# Autodesk Inventor assembly: OBG-Elektronik
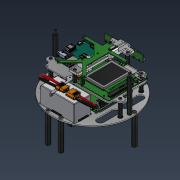
[picture p0: Inventor's stored thumbnail of the model, 180x180]
Saved by Autodesk Inventor 2022.1 (Build 261234020, 234B)
## iProperties
Part Number: OBG-Elektronik
Material: Generisch
Document SubType Name: Assembly
Designer: rYan
Mass: 726.974 g
Surface Area: 2264.16 cm^2
Volume: 285.444 cm^3
Density: 2.54682 g/cm^3
Author: rYan
## Documents named in this file (16)
- D:\TIGERsGIT\Hardware\mechanik\2020\Inventor\Robot\Electronics\OBG-Elektronik.iam
- D:\TIGERsGIT\Hardware\mechanik\2020\Inventor\Robot\Electronics\Mittelplatte.ipt
- D:\TIGERsGIT\Hardware\mechanik\2019\Inventor\Kaufteile\Abstandsbolzen Typ A.ipt
- D:\TIGERsGIT\Hardware\mechanik\2020\Inventor\Inhaltscenter\de-DE\DIN 7984\DIN 7984 - M4 x 6.ipt
- D:\TIGERsGIT\Hardware\mechanik\2020\Inventor\Purchased Parts\Abstandsbolzen Typ A M4 60mm SW8.ipt
- D:\TIGERsGIT\Hardware\mechanik\2020\Inventor\Robot\Electronics\MG-Powerboard.iam
- D:\TIGERsGIT\Hardware\mechanik\2019\Inventor\Kaufteile\Abstandsbolzen Typ B.ipt
- D:\TIGERsGIT\Hardware\mechanik\2020\Inventor\Robot\Electronics\UBG-Compute Layer.iam
- D:\TIGERsGIT\Hardware\mechanik\2020\Inventor\Purchased Parts\Abstandsbolzen Typ B M4 70mm.ipt
- D:\TIGERsGIT\Hardware\mechanik\2020\Inventor\Purchased Parts\MG-Akku 6S1P.iam
- D:\TIGERsGIT\Hardware\mechanik\2020\Inventor\Robot\Electronics\Akkuhalter.ipt
- D:\TIGERsGIT\Hardware\mechanik\2020\Inventor\Purchased Parts\Gummitülle 3mm.ipt
- D:\TIGERsGIT\Hardware\mechanik\2020\Inventor\Inhaltscenter\de-DE\ISO 4762(2)\ISO 4762 - M2 x 6ISO.ipt
- D:\TIGERsGIT\Hardware\mechanik\2020\Inventor\Robot\Electronics\UBG-Kamera mit Halter geneigt.iam
- D:\TIGERsGIT\Hardware\mechanik\2020\Inventor\Inhaltscenter\de-DE\DIN 7984\DIN 7984 - M3 x 5.ipt
- D:\TIGERsGIT\Hardware\mechanik\2020\Inventor\Inhaltscenter\de-DE\ISO 10642(1)\ISO 10642 - M3 x  8.ipt
## Components (32 placed, 13 different names)
1. Mittelplatte:1 — Einfügen:1, Einfügen:3, Einfügen:4, Einfügen:6, Einfügen:7, Einfügen:8, Fluchtend:1, Fluchtend:2, Fluchtend:3, Passend:19, Einfügen:34, Einfügen:36, Einfügen:42, Einfügen:43, Einfügen:44, Einfügen:45, Einfügen:55, Passend:25, Einfügen:56, Einfügen:57, Einfügen:58, Einfügen:59, Einfügen:64, Einfügen:65, Einfügen:66, Einfügen:67, Passend:28, Passend:29, Passend:30, Einfügen:68, Passend:34, Einfügen:69, Einfügen:70
2. Abstandsbolzen Typ A M4 60mm SW8:1 — Einfügen:3
3. Abstandsbolzen Typ A M4 60mm SW8:2 — Einfügen:1
4. Abstandsbolzen Typ A M4 60mm SW8:4 — Einfügen:4
5. Abstandsbolzen Typ A M4 60mm SW8:6 — Einfügen:6
6. DIN 7984 M4 x 6:1 — Einfügen:7
7. DIN 7984 M4 x 6:2 — Einfügen:8
8. MG-Powerboard:1 [sub-assembly] — Einfügen:55, Passend:25
9. UBG-Compute Layer:1 [sub-assembly] — Passend:19, Einfügen:50
10. DIN 7984 M4 x 6:4 — Einfügen:34
11. DIN 7984 M4 x 6:6 — Einfügen:36
12. Abstandsbolzen Typ B M4 70mm:5 — Einfügen:42
13. Abstandsbolzen Typ B M4 70mm:6 — Einfügen:43
14. DIN 7984 M4 x 6:7 — Einfügen:44
15. DIN 7984 M4 x 6:8 — Einfügen:45
16. MG-Akku 6S1P:1 [sub-assembly] — Passend:31, Passend:32, Passend:33
17. Akkuhalter:1 — Passend:28, Passend:29, Passend:30, Passend:31, Passend:32, Passend:33
18. Gummitülle 3mm:1 — Einfügen:64, Einfügen:73
19. Gummitülle 3mm:2 — Einfügen:50, Einfügen:65, Einfügen:74
20. Gummitülle 3mm:3 — Einfügen:66, Einfügen:72
21. Gummitülle 3mm:4 — Einfügen:67, Einfügen:71
22. ISO 4762 M2 x 6:1 — Einfügen:58
23. ISO 4762 M2 x 6:2 — Einfügen:59
24. ISO 4762 M2 x 6:3 — Einfügen:57
25. ISO 4762 M2 x 6:4 — Einfügen:56
26. DIN 7984 M3 x 5:4 — Einfügen:70
27. DIN 7984 M3 x 5:5 — Einfügen:69
28. UBG-Kamera mit Halter geneigt:1 [sub-assembly] — Einfügen:68, Passend:34
29. ISO 10642 M3 x  8:1 — Einfügen:73
30. ISO 10642 M3 x  8:2 — Einfügen:74
31. ISO 10642 M3 x  8:3 — Einfügen:72
32. ISO 10642 M3 x  8:4 — Einfügen:71
## Relationships (41: Insert 29, Mate 9, Flush 3)
- Einfügen:1 [Insert]: Mittelplatte:1 ↔ Abstandsbolzen Typ A M4 60mm SW8:2
- Einfügen:3 [Insert]: Mittelplatte:1 ↔ Abstandsbolzen Typ A M4 60mm SW8:1
- Einfügen:4 [Insert]: Mittelplatte:1 ↔ Abstandsbolzen Typ A M4 60mm SW8:4
- Einfügen:6 [Insert]: Mittelplatte:1 ↔ Abstandsbolzen Typ A M4 60mm SW8:6
- Einfügen:7 [Insert]: Mittelplatte:1 ↔ DIN 7984 M4 x 6:1
- Einfügen:8 [Insert]: Mittelplatte:1 ↔ DIN 7984 M4 x 6:2
- Fluchtend:1 [Flush]: Mittelplatte:1
- Fluchtend:2 [Flush]: Mittelplatte:1
- Fluchtend:3 [Flush]: Mittelplatte:1
- Passend:19 [Mate]: Mittelplatte:1 ↔ UBG-Compute Layer:1
- Einfügen:34 [Insert]: Mittelplatte:1 ↔ DIN 7984 M4 x 6:4
- Einfügen:36 [Insert]: Mittelplatte:1 ↔ DIN 7984 M4 x 6:6
- Einfügen:42 [Insert]: Mittelplatte:1 ↔ Abstandsbolzen Typ B M4 70mm:5
- Einfügen:43 [Insert]: Mittelplatte:1 ↔ Abstandsbolzen Typ B M4 70mm:6
- Einfügen:44 [Insert]: Mittelplatte:1 ↔ DIN 7984 M4 x 6:7
- Einfügen:45 [Insert]: Mittelplatte:1 ↔ DIN 7984 M4 x 6:8
- Einfügen:50 [Insert]: UBG-Compute Layer:1 ↔ Gummitülle 3mm:2
- Einfügen:55 [Insert]: Mittelplatte:1 ↔ MG-Powerboard:1
- Passend:25 [Mate]: Mittelplatte:1 ↔ MG-Powerboard:1
- Einfügen:56 [Insert]: Mittelplatte:1 ↔ ISO 4762 M2 x 6:4
- Einfügen:57 [Insert]: Mittelplatte:1 ↔ ISO 4762 M2 x 6:3
- Einfügen:58 [Insert]: Mittelplatte:1 ↔ ISO 4762 M2 x 6:1
- Einfügen:59 [Insert]: Mittelplatte:1 ↔ ISO 4762 M2 x 6:2
- Einfügen:64 [Insert]: Mittelplatte:1 ↔ Gummitülle 3mm:1
- Einfügen:65 [Insert]: Mittelplatte:1 ↔ Gummitülle 3mm:2
- Einfügen:66 [Insert]: Mittelplatte:1 ↔ Gummitülle 3mm:3
- Einfügen:67 [Insert]: Mittelplatte:1 ↔ Gummitülle 3mm:4
- Passend:28 [Mate] (0.1 mm): Mittelplatte:1 ↔ Akkuhalter:1
- Passend:29 [Mate] (0.1 mm): Mittelplatte:1 ↔ Akkuhalter:1
- Passend:30 [Mate]: Mittelplatte:1 ↔ Akkuhalter:1
- Passend:31 [Mate]: MG-Akku 6S1P:1 ↔ Akkuhalter:1
- Passend:32 [Mate] (0.5 mm): MG-Akku 6S1P:1 ↔ Akkuhalter:1
- Passend:33 [Mate] (1 mm): MG-Akku 6S1P:1 ↔ Akkuhalter:1
- Einfügen:68 [Insert]: Mittelplatte:1 ↔ UBG-Kamera mit Halter geneigt:1
- Passend:34 [Mate]: Mittelplatte:1 ↔ UBG-Kamera mit Halter geneigt:1
- Einfügen:69 [Insert]: Mittelplatte:1 ↔ DIN 7984 M3 x 5:5
- Einfügen:70 [Insert]: Mittelplatte:1 ↔ DIN 7984 M3 x 5:4
- Einfügen:71 [Insert] (-0.5 mm): Gummitülle 3mm:4 ↔ ISO 10642 M3 x  8:4
- Einfügen:72 [Insert] (-0.5 mm): Gummitülle 3mm:3 ↔ ISO 10642 M3 x  8:3
- Einfügen:73 [Insert] (-0.5 mm): Gummitülle 3mm:1 ↔ ISO 10642 M3 x  8:1
- Einfügen:74 [Insert] (-0.5 mm): Gummitülle 3mm:2 ↔ ISO 10642 M3 x  8:2
